# Autodesk Inventor assembly: 2307-0006-0028 bevel gear
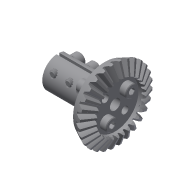
[picture p0: Inventor's stored thumbnail of the model, 180x180]
Saved by Autodesk Inventor 2018 (Build 220112000, 112)
## iProperties
Created: 2019-01-13
Part Number: 2307-0006-0028 bevel gear
Document SubType Name: Assembly
Designer: ball
Author: ball
## Documents named in this file (4)
- C:\FTC\FTC8863CAD\GoBilda\2307 parts\2307-0006-0028 bevel gear.iam
- C:\FTC\FTC8863CAD\GoBilda\2307 parts\2307-0006-0028.ipt
- C:\FTC\FTC8863CAD\GoBilda\1306 Parts\1306-0016-1006 assembly.ipt
- C:\FTC\FTC8863CAD\GoBilda\2800 Parts\2800-0004-0008.ipt
## Components (4 placed, 3 different names)
1. 2307-0006-0028:1 — Mate:1, Mate:2, Mate:3, Mate:4, Mate:5, Mate:6, Mate:7
2. 1306-0016-1006 assembly:1 — Mate:1, Mate:2, Mate:3
3. 2800-0004-0008:1 — Mate:4, Mate:5
4. 2800-0004-0008:2 — Mate:6, Mate:7
## Relationships (7: Mate 7)
- Mate:1: 2307-0006-0028:1 ↔ 1306-0016-1006 assembly:1
- Mate:2: 2307-0006-0028:1 ↔ 1306-0016-1006 assembly:1
- Mate:3: 2307-0006-0028:1 ↔ 1306-0016-1006 assembly:1
- Mate:4: 2307-0006-0028:1 ↔ 2800-0004-0008:1
- Mate:5: 2307-0006-0028:1 ↔ 2800-0004-0008:1
- Mate:6: 2307-0006-0028:1 ↔ 2800-0004-0008:2
- Mate:7: 2307-0006-0028:1 ↔ 2800-0004-0008:2
